# Autodesk Inventor assembly: ASY MSC 500 BELLY
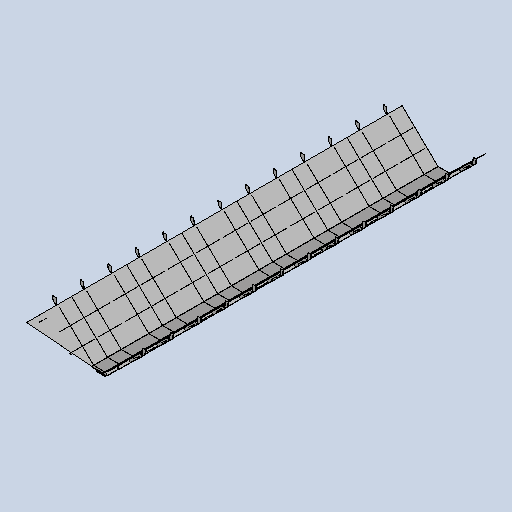
[picture p0: Inventor's stored thumbnail of the model, 512x512]
Saved by Autodesk Inventor 2025 (Build 290162010, 162A)
## iProperties
Created: 2024-07-22
Part Number: ASY MSC 500 BELLY
Document SubType Name: Assembly
Designer: pokla
Stock Number: ASY МОО 500 брюхо
Author: pokla
## Documents named in this file (7)
- C:\Users\pokla\Documents\Inventor\Отстойник осветлитель\Manturovo_Se-clar-Gleb\ASY MSC 500 BELLY.iam
- C:\Users\pokla\Documents\Inventor\Отстойник осветлитель\Manturovo_Se-clar-Gleb\MSC 501 sheet belly main.ipt
- C:\Users\pokla\Documents\Inventor\Отстойник осветлитель\Manturovo_Se-clar-Gleb\MSC 502 sheet belly-neck.ipt
- C:\Users\pokla\Documents\Inventor\Отстойник осветлитель\Manturovo_Se-clar-Gleb\MSC 504 stringer board belly.ipt
- C:\Users\pokla\Documents\Inventor\Отстойник осветлитель\Manturovo_Se-clar-Gleb\MSC 503 rib belly.ipt
- C:\Users\pokla\Documents\Inventor\Отстойник осветлитель\Manturovo_Se-clar-Gleb\MSC 505 STRINGER BOARD BELLY FACE.ipt
- C:\Users\pokla\Documents\Inventor\Отстойник осветлитель\Manturovo_Se-clar-Gleb\MSC 506 STRINGER BOARD BELLY.ipt
## Components (87 placed, 6 different names)
1. MSC 501 sheet belly main.ipt:1
2. MSC 501 sheet belly main.ipt:2
3. MSC 501 sheet belly main.ipt:3
4. MSC 502 sheet belly-neck.ipt:1 — Rigid:24
5. MSC 501 sheet belly main.ipt:4
6. MSC 501 sheet belly main.ipt:5 — Rigid:24
7. MSC 501 sheet belly main.ipt:6 — Mate:4, Mate:5, Mate:6, Mate:7, Flush:1, Mate:9, Mate:10, Flush:2, Mate:11, Mate:12
8. MSC 503 rib belly.ipt:1 — Rigid:17, Rigid:20, Rigid:21, Mate:13, Mate:15, Mate:16, Mate:17
9. MSC 503 rib belly.ipt:2 — Rigid:18, Rigid:19, Mate:11, Mate:12, Mate:13, Mate:14, Mate:18, Mate:19
10. MSC 504 stringer board belly.ipt:1 — Rigid:21, Flush:2
11. MSC 504 stringer board belly.ipt:2 — Rigid:20
12. MSC 504 stringer board belly.ipt:3 — Rigid:19
13. MSC 504 stringer board belly.ipt:4 — Rigid:18
14. MSC 505 STRINGER BOARD BELLY FACE.ipt:1 — Rigid:25
15. MSC 505 STRINGER BOARD BELLY FACE.ipt:2 — Rigid:26
16. MSC 505 STRINGER BOARD BELLY FACE.ipt:3
17. MSC 505 STRINGER BOARD BELLY FACE.ipt:4 — Rigid:28
18. MSC 506 STRINGER BOARD BELLY.ipt:25 — Mate:14, Mate:18, Mate:19, Rigid:29
19. MSC 506 STRINGER BOARD BELLY.ipt:26 — Mate:15, Mate:16, Mate:17, Rigid:30
20. MSC 504 stringer board belly.ipt:5
21. MSC 504 stringer board belly.ipt:6
22. MSC 504 stringer board belly.ipt:7
23. MSC 504 stringer board belly.ipt:8
24. MSC 504 stringer board belly.ipt:9
25. MSC 504 stringer board belly.ipt:10
26. MSC 504 stringer board belly.ipt:11
27. MSC 504 stringer board belly.ipt:12
28. MSC 504 stringer board belly.ipt:13
29. MSC 504 stringer board belly.ipt:14
30. MSC 504 stringer board belly.ipt:15
31. MSC 504 stringer board belly.ipt:16
32. MSC 504 stringer board belly.ipt:17
33. MSC 504 stringer board belly.ipt:18
34. MSC 504 stringer board belly.ipt:19
35. MSC 504 stringer board belly.ipt:20
36. MSC 504 stringer board belly.ipt:21 — Rigid:28
37. MSC 504 stringer board belly.ipt:22
38. MSC 504 stringer board belly.ipt:23 — Rigid:25
39. MSC 504 stringer board belly.ipt:24 — Rigid:26
40. MSC 503 rib belly.ipt:3 — Mate:6, Mate:7, Mate:8, Rigid:17
41. MSC 503 rib belly.ipt:4 — Mate:4, Mate:5, Mate:8
42. MSC 506 STRINGER BOARD BELLY.ipt:1 — Rigid:30
43. MSC 506 STRINGER BOARD BELLY.ipt:2 — Rigid:29
44. MSC 503 rib belly.ipt:5
45. MSC 503 rib belly.ipt:6
46. MSC 506 STRINGER BOARD BELLY.ipt:3
47. MSC 506 STRINGER BOARD BELLY.ipt:4
48. MSC 503 rib belly.ipt:7
49. MSC 503 rib belly.ipt:8
50. MSC 506 STRINGER BOARD BELLY.ipt:5
51. MSC 506 STRINGER BOARD BELLY.ipt:6
52. MSC 503 rib belly.ipt:9
53. MSC 503 rib belly.ipt:10
54. MSC 506 STRINGER BOARD BELLY.ipt:7
55. MSC 506 STRINGER BOARD BELLY.ipt:8
56. MSC 503 rib belly.ipt:11
57. MSC 503 rib belly.ipt:12
58. MSC 506 STRINGER BOARD BELLY.ipt:9
59. MSC 506 STRINGER BOARD BELLY.ipt:10
60. MSC 503 rib belly.ipt:13
61. MSC 503 rib belly.ipt:14
62. MSC 506 STRINGER BOARD BELLY.ipt:11
63. MSC 506 STRINGER BOARD BELLY.ipt:12
64. MSC 503 rib belly.ipt:15
65. MSC 503 rib belly.ipt:16
66. MSC 506 STRINGER BOARD BELLY.ipt:13
67. MSC 506 STRINGER BOARD BELLY.ipt:14
68. MSC 503 rib belly.ipt:17
69. MSC 503 rib belly.ipt:18
70. MSC 506 STRINGER BOARD BELLY.ipt:15
71. MSC 506 STRINGER BOARD BELLY.ipt:16
72. MSC 503 rib belly.ipt:19
73. MSC 503 rib belly.ipt:20
74. MSC 506 STRINGER BOARD BELLY.ipt:17
75. MSC 506 STRINGER BOARD BELLY.ipt:18
76. MSC 503 rib belly.ipt:21
77. MSC 503 rib belly.ipt:22
78. MSC 506 STRINGER BOARD BELLY.ipt:19
79. MSC 506 STRINGER BOARD BELLY.ipt:20
80. MSC 503 rib belly.ipt:23
81. MSC 503 rib belly.ipt:24
82. MSC 506 STRINGER BOARD BELLY.ipt:21
83. MSC 506 STRINGER BOARD BELLY.ipt:22
84. MSC 503 rib belly.ipt:25
85. MSC 503 rib belly.ipt:26
86. MSC 506 STRINGER BOARD BELLY.ipt:23
87. MSC 506 STRINGER BOARD BELLY.ipt:24
## Component patterns: (5 elements, first: MSC 504 stringer board belly.ipt:5 + MSC 504 stringer board belly.ipt:6 + MSC 504 stringer board belly.ipt:7 + MSC 504 stringer board belly.ipt:8), (12 elements, first: MSC 503 rib belly.ipt:3 + MSC 503 rib belly.ipt:4 + MSC 506 STRINGER BOARD BELLY.ipt:1 + MSC 506 STRINGER BOARD BELLY.ipt:2)
## Relationships (38: WeldJoint 20, Mate 16, Flush 2)
- [WeldJoint]: MSC 501 sheet belly main.ipt:1 ↔ MSC 501 sheet belly main.ipt:2
- [WeldJoint]: MSC 501 sheet belly main.ipt:1 ↔ MSC 501 sheet belly main.ipt:3
- [WeldJoint]: MSC 501 sheet belly main.ipt:4 ↔ MSC 501 sheet belly main.ipt:5
- [WeldJoint]: MSC 501 sheet belly main.ipt:3 ↔ MSC 501 sheet belly main.ipt:4
- [WeldJoint]: MSC 501 sheet belly main.ipt:2 ↔ MSC 501 sheet belly main.ipt:6
- [WeldJoint]: MSC 504 stringer board belly.ipt:3 ↔ MSC 504 stringer board belly.ipt:5
- [WeldJoint]: MSC 504 stringer board belly.ipt:4 ↔ MSC 504 stringer board belly.ipt:6
- [WeldJoint]: MSC 504 stringer board belly.ipt:2 ↔ MSC 504 stringer board belly.ipt:7
- [WeldJoint]: MSC 504 stringer board belly.ipt:1 ↔ MSC 504 stringer board belly.ipt:8
- Mate:4: MSC 501 sheet belly main.ipt:6 ↔ MSC 503 rib belly.ipt:4
- Mate:5: MSC 501 sheet belly main.ipt:6 ↔ MSC 503 rib belly.ipt:4
- Mate:6: MSC 501 sheet belly main.ipt:6 ↔ MSC 503 rib belly.ipt:3
- Mate:7: MSC 501 sheet belly main.ipt:6 ↔ MSC 503 rib belly.ipt:3
- Mate:8: MSC 503 rib belly.ipt:3 ↔ MSC 503 rib belly.ipt:4
- Flush:1: MSC 501 sheet belly main.ipt:6
- Mate:9: MSC 501 sheet belly main.ipt:6
- Mate:10: MSC 501 sheet belly main.ipt:6
- Rigid:17 [WeldJoint] (490 mm): MSC 503 rib belly.ipt:1 ↔ MSC 503 rib belly.ipt:3
- Rigid:18 [WeldJoint]: MSC 503 rib belly.ipt:2 ↔ MSC 504 stringer board belly.ipt:4
- Rigid:19 [WeldJoint]: MSC 503 rib belly.ipt:2 ↔ MSC 504 stringer board belly.ipt:3
- Rigid:20 [WeldJoint]: MSC 503 rib belly.ipt:1 ↔ MSC 504 stringer board belly.ipt:2
- Rigid:21 [WeldJoint]: MSC 503 rib belly.ipt:1 ↔ MSC 504 stringer board belly.ipt:1
- Flush:2: MSC 501 sheet belly main.ipt:6 ↔ MSC 504 stringer board belly.ipt:1
- Mate:11: MSC 501 sheet belly main.ipt:6 ↔ MSC 503 rib belly.ipt:2
- Mate:12: MSC 501 sheet belly main.ipt:6 ↔ MSC 503 rib belly.ipt:2
- Mate:13: MSC 503 rib belly.ipt:1 ↔ MSC 503 rib belly.ipt:2
- Rigid:24 [WeldJoint]: MSC 502 sheet belly-neck.ipt:1 ↔ MSC 501 sheet belly main.ipt:5
- Rigid:25 [WeldJoint]: MSC 505 STRINGER BOARD BELLY FACE.ipt:1 ↔ MSC 504 stringer board belly.ipt:23
- Rigid:26 [WeldJoint]: MSC 505 STRINGER BOARD BELLY FACE.ipt:2 ↔ MSC 504 stringer board belly.ipt:24
- Rigid:28 [WeldJoint]: MSC 505 STRINGER BOARD BELLY FACE.ipt:4 ↔ MSC 504 stringer board belly.ipt:21
- Mate:14: MSC 503 rib belly.ipt:2 ↔ MSC 506 STRINGER BOARD BELLY.ipt:25
- Mate:15: MSC 503 rib belly.ipt:1 ↔ MSC 506 STRINGER BOARD BELLY.ipt:26
- Mate:16: MSC 503 rib belly.ipt:1 ↔ MSC 506 STRINGER BOARD BELLY.ipt:26
- Mate:17 (-20 mm): MSC 503 rib belly.ipt:1 ↔ MSC 506 STRINGER BOARD BELLY.ipt:26
- Mate:18: MSC 503 rib belly.ipt:2 ↔ MSC 506 STRINGER BOARD BELLY.ipt:25
- Mate:19 (-20 mm): MSC 503 rib belly.ipt:2 ↔ MSC 506 STRINGER BOARD BELLY.ipt:25
- Rigid:29 [WeldJoint] (-490 mm): MSC 506 STRINGER BOARD BELLY.ipt:25 ↔ MSC 506 STRINGER BOARD BELLY.ipt:2
- Rigid:30 [WeldJoint] (-490 mm): MSC 506 STRINGER BOARD BELLY.ipt:26 ↔ MSC 506 STRINGER BOARD BELLY.ipt:1
